# Autodesk Inventor assembly: CycloidalGearBoxAssemblyV1
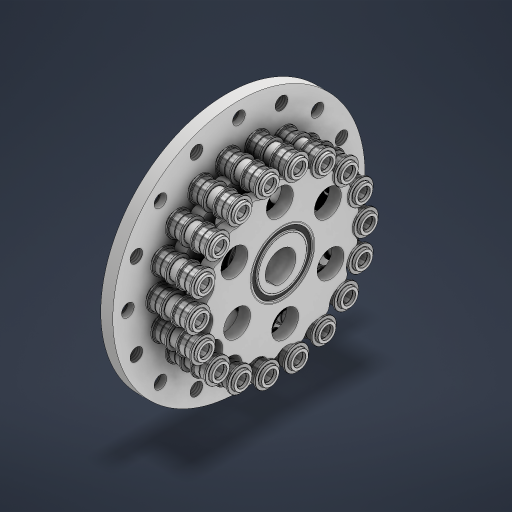
[picture p0: Inventor's stored thumbnail of the model, 512x512]
Saved by Autodesk Inventor 2024 (Build 280153000, 153)
## iProperties
Created: 2024-01-31
Part Number: CycloidalGearBoxAssemblyV1
Document SubType Name: Assembly
Designer: avsar
Author: avsar
## Documents named in this file (10)
- C:\Users\avsar\Documents\Inventor\RCR_Arm\Arm_V4\CycloidalGearBoxes\StageOneGearBox\CycloidalGearBoxAssemblyV1.iam
- C:\Users\avsar\Documents\Inventor\RCR_Arm\Arm_V4\CycloidalGearBoxes\StageOneGearBox\HousingFaceInput.ipt
- C:\Users\avsar\Documents\Inventor\RCR_Arm\Arm_V4\CycloidalGearBoxes\StageOneGearBox\Gearbox_MainBody.ipt
- C:\Users\avsar\Documents\Inventor\RCR_Arm\COTS\Motion\Bearings\Flanged Bearings\4x7x2.5mm Flanged Ball Bearing.ipt
- C:\Users\avsar\Documents\Inventor\RCR_Arm\COTS\ISO Standard Hardware\Spacers and Shims\4mm ID x 6mm OD Spacers\(1mm legnth) 4mm ID x 6mm OD Spacer.ipt
- C:\Users\avsar\Documents\Inventor\RCR_Arm\COTS\ISO Standard Hardware\Spacers and Shims\4mm ID x 6mm OD Spacers\(3mm legnth) 4mm ID x 6mm OD Spacer.ipt
- C:\Users\avsar\Documents\Inventor\RCR_Arm\Arm_V4\CycloidalGearBoxes\StageOneGearBox\RollerBearingShaft.ipt
- C:\Users\avsar\Documents\Inventor\RCR_Arm\Arm_V4\CycloidalGearBoxes\StageOneGearBox\CycloidalDisk.ipt
- C:\Users\avsar\Documents\Inventor\RCR_Arm\Arm_V4\CycloidalGearBoxes\StageOneGearBox\EccentricBearingShaft.ipt
- C:\Users\avsar\Documents\Inventor\RCR_Arm\COTS\Motion\Bearings\Standard Bearings\16mm ID x 22mm OD x 4mm Thickness Ball Bearing.ipt
## Components (169 placed, 9 different names)
1. HousingFaceInput:1 — Mate:1, Mate:2, Mate:3, Mate:4, Mate:5, Mate:7, Mate:75, Mate:76, Mate:93, Mate:94, Mate:111, Mate:112, Mate:129, Mate:130, Mate:147, Mate:148, Mate:165, Mate:166, Mate:183, Mate:184, Mate:201, Mate:202, Mate:219, Mate:220, Mate:237, Mate:238, Mate:255, Mate:256, Mate:273, Mate:274, Mate:291, Mate:292, Mate:309, Mate:310, Mate:327, Mate:328, Mate:345, Mate:346, Mate:363, Mate:364
2. Gearbox_MainBody:1 — Mate:1, Mate:2, Mate:3
3. (1mm legnth) 4mm ID x 6mm OD Spacer:1 — Mate:4, Mate:5, Mate:6, Mate:58
4. 4x7x2.5mm Flanged Ball Bearing:5 — Mate:10, Mate:11, Mate:12, Mate:13
5. RollerBearingShaft:2 — Mate:8, Mate:9, Mate:10, Mate:11
6. 4x7x2.5mm Flanged Ball Bearing:4 — Mate:6, Mate:7, Mate:8, Mate:9, Mate:58
7. (1mm legnth) 4mm ID x 6mm OD Spacer:2 — Mate:20, Mate:21
8. RollerBearingShaft:1 — Mate:16, Mate:17, Mate:18, Mate:19
9. 4x7x2.5mm Flanged Ball Bearing:2 — Mate:14, Mate:15, Mate:16, Mate:17
10. (3mm legnth) 4mm ID x 6mm OD Spacer:1 — Mate:12, Mate:13, Mate:14, Mate:15
11. 4x7x2.5mm Flanged Ball Bearing:1 — Mate:18, Mate:19, Mate:20, Mate:21
12. (1mm legnth) 4mm ID x 6mm OD Spacer:3 — Mate:76
13. (1mm legnth) 4mm ID x 6mm OD Spacer:4 — Mate:75
14. 4x7x2.5mm Flanged Ball Bearing:6
15. RollerBearingShaft:3
16. 4x7x2.5mm Flanged Ball Bearing:7 — Tangent:2
17. 4x7x2.5mm Flanged Ball Bearing:8
18. RollerBearingShaft:4
19. 4x7x2.5mm Flanged Ball Bearing:9
20. (3mm legnth) 4mm ID x 6mm OD Spacer:2
21. (1mm legnth) 4mm ID x 6mm OD Spacer:5 — Mate:94
22. (1mm legnth) 4mm ID x 6mm OD Spacer:6 — Mate:93
23. 4x7x2.5mm Flanged Ball Bearing:10
24. RollerBearingShaft:5
25. 4x7x2.5mm Flanged Ball Bearing:11
26. 4x7x2.5mm Flanged Ball Bearing:12
27. RollerBearingShaft:6
28. 4x7x2.5mm Flanged Ball Bearing:13
29. (3mm legnth) 4mm ID x 6mm OD Spacer:3
30. (1mm legnth) 4mm ID x 6mm OD Spacer:7 — Mate:112
31. (1mm legnth) 4mm ID x 6mm OD Spacer:8 — Mate:111
32. 4x7x2.5mm Flanged Ball Bearing:14
33. RollerBearingShaft:7
34. 4x7x2.5mm Flanged Ball Bearing:15
35. 4x7x2.5mm Flanged Ball Bearing:16 — Tangent:3
36. RollerBearingShaft:8
37. 4x7x2.5mm Flanged Ball Bearing:17
38. (3mm legnth) 4mm ID x 6mm OD Spacer:4
39. (1mm legnth) 4mm ID x 6mm OD Spacer:9
40. (1mm legnth) 4mm ID x 6mm OD Spacer:10 — Mate:129
41. 4x7x2.5mm Flanged Ball Bearing:18
42. RollerBearingShaft:9
43. 4x7x2.5mm Flanged Ball Bearing:19
44. 4x7x2.5mm Flanged Ball Bearing:20 — Mate:130
45. RollerBearingShaft:10
46. 4x7x2.5mm Flanged Ball Bearing:21
47. (3mm legnth) 4mm ID x 6mm OD Spacer:5
48. (1mm legnth) 4mm ID x 6mm OD Spacer:11
49. (1mm legnth) 4mm ID x 6mm OD Spacer:12 — Mate:147
50. 4x7x2.5mm Flanged Ball Bearing:22 — Mate:365, Tangent:1
51. RollerBearingShaft:11
52. 4x7x2.5mm Flanged Ball Bearing:23
53. 4x7x2.5mm Flanged Ball Bearing:24 — Mate:148
54. RollerBearingShaft:12
55. 4x7x2.5mm Flanged Ball Bearing:25 — Mate:366
56. (3mm legnth) 4mm ID x 6mm OD Spacer:6
57. (1mm legnth) 4mm ID x 6mm OD Spacer:13
58. (1mm legnth) 4mm ID x 6mm OD Spacer:14 — Mate:165
59. 4x7x2.5mm Flanged Ball Bearing:26
60. RollerBearingShaft:13
61. 4x7x2.5mm Flanged Ball Bearing:27
62. 4x7x2.5mm Flanged Ball Bearing:28 — Mate:166
63. RollerBearingShaft:14
64. 4x7x2.5mm Flanged Ball Bearing:29
65. (3mm legnth) 4mm ID x 6mm OD Spacer:7
66. (1mm legnth) 4mm ID x 6mm OD Spacer:15
67. (1mm legnth) 4mm ID x 6mm OD Spacer:16 — Mate:183
68. 4x7x2.5mm Flanged Ball Bearing:30
69. RollerBearingShaft:15
70. 4x7x2.5mm Flanged Ball Bearing:31
71. 4x7x2.5mm Flanged Ball Bearing:32 — Mate:184
72. RollerBearingShaft:16
73. 4x7x2.5mm Flanged Ball Bearing:33
74. (3mm legnth) 4mm ID x 6mm OD Spacer:8
75. (1mm legnth) 4mm ID x 6mm OD Spacer:17
76. (1mm legnth) 4mm ID x 6mm OD Spacer:18 — Mate:201
77. 4x7x2.5mm Flanged Ball Bearing:34
78. RollerBearingShaft:17
79. 4x7x2.5mm Flanged Ball Bearing:35
80. 4x7x2.5mm Flanged Ball Bearing:36 — Mate:202
81. RollerBearingShaft:18
82. 4x7x2.5mm Flanged Ball Bearing:37
83. (3mm legnth) 4mm ID x 6mm OD Spacer:9
84. (1mm legnth) 4mm ID x 6mm OD Spacer:19
85. (1mm legnth) 4mm ID x 6mm OD Spacer:20 — Mate:219
86. 4x7x2.5mm Flanged Ball Bearing:38
87. RollerBearingShaft:19
88. 4x7x2.5mm Flanged Ball Bearing:39
89. 4x7x2.5mm Flanged Ball Bearing:40 — Mate:220
90. RollerBearingShaft:20
91. 4x7x2.5mm Flanged Ball Bearing:41
92. (3mm legnth) 4mm ID x 6mm OD Spacer:10
93. (1mm legnth) 4mm ID x 6mm OD Spacer:21
94. (1mm legnth) 4mm ID x 6mm OD Spacer:22 — Mate:237
95. 4x7x2.5mm Flanged Ball Bearing:42
96. RollerBearingShaft:21
97. 4x7x2.5mm Flanged Ball Bearing:43
98. 4x7x2.5mm Flanged Ball Bearing:44 — Mate:238
99. RollerBearingShaft:22
100. 4x7x2.5mm Flanged Ball Bearing:45
101. (3mm legnth) 4mm ID x 6mm OD Spacer:11
102. (1mm legnth) 4mm ID x 6mm OD Spacer:23
103. (1mm legnth) 4mm ID x 6mm OD Spacer:24 — Mate:255
104. 4x7x2.5mm Flanged Ball Bearing:46 — Mate:256
105. RollerBearingShaft:23
106. 4x7x2.5mm Flanged Ball Bearing:47
107. 4x7x2.5mm Flanged Ball Bearing:48
108. RollerBearingShaft:24
109. 4x7x2.5mm Flanged Ball Bearing:49
110. (3mm legnth) 4mm ID x 6mm OD Spacer:12
111. (1mm legnth) 4mm ID x 6mm OD Spacer:25
112. (1mm legnth) 4mm ID x 6mm OD Spacer:26 — Mate:273
113. 4x7x2.5mm Flanged Ball Bearing:50
114. RollerBearingShaft:25
115. 4x7x2.5mm Flanged Ball Bearing:51
116. 4x7x2.5mm Flanged Ball Bearing:52 — Mate:274
117. RollerBearingShaft:26
118. 4x7x2.5mm Flanged Ball Bearing:53
119. (3mm legnth) 4mm ID x 6mm OD Spacer:13
120. (1mm legnth) 4mm ID x 6mm OD Spacer:27
121. (1mm legnth) 4mm ID x 6mm OD Spacer:28 — Mate:291
122. 4x7x2.5mm Flanged Ball Bearing:54
123. RollerBearingShaft:27
124. 4x7x2.5mm Flanged Ball Bearing:55
125. 4x7x2.5mm Flanged Ball Bearing:56 — Mate:292
126. RollerBearingShaft:28
127. 4x7x2.5mm Flanged Ball Bearing:57
128. (3mm legnth) 4mm ID x 6mm OD Spacer:14
129. (1mm legnth) 4mm ID x 6mm OD Spacer:29
130. (1mm legnth) 4mm ID x 6mm OD Spacer:30 — Mate:309
131. 4x7x2.5mm Flanged Ball Bearing:58
132. RollerBearingShaft:29
133. 4x7x2.5mm Flanged Ball Bearing:59
134. 4x7x2.5mm Flanged Ball Bearing:60 — Mate:310
135. RollerBearingShaft:30
136. 4x7x2.5mm Flanged Ball Bearing:61
137. (3mm legnth) 4mm ID x 6mm OD Spacer:15
138. (1mm legnth) 4mm ID x 6mm OD Spacer:31
139. (1mm legnth) 4mm ID x 6mm OD Spacer:32 — Mate:327
140. 4x7x2.5mm Flanged Ball Bearing:62
141. RollerBearingShaft:31
142. 4x7x2.5mm Flanged Ball Bearing:63
143. 4x7x2.5mm Flanged Ball Bearing:64 — Mate:328
144. RollerBearingShaft:32
145. 4x7x2.5mm Flanged Ball Bearing:65
146. (3mm legnth) 4mm ID x 6mm OD Spacer:16
147. (1mm legnth) 4mm ID x 6mm OD Spacer:33
148. (1mm legnth) 4mm ID x 6mm OD Spacer:34 — Mate:345
149. 4x7x2.5mm Flanged Ball Bearing:66
150. RollerBearingShaft:33
151. 4x7x2.5mm Flanged Ball Bearing:67
152. 4x7x2.5mm Flanged Ball Bearing:68 — Mate:346, Tangent:4
153. RollerBearingShaft:34
154. 4x7x2.5mm Flanged Ball Bearing:69
155. (3mm legnth) 4mm ID x 6mm OD Spacer:17
156. (1mm legnth) 4mm ID x 6mm OD Spacer:35
157. (1mm legnth) 4mm ID x 6mm OD Spacer:36 — Mate:363
158. 4x7x2.5mm Flanged Ball Bearing:70
159. RollerBearingShaft:35
160. 4x7x2.5mm Flanged Ball Bearing:71
161. 4x7x2.5mm Flanged Ball Bearing:72 — Mate:364
162. RollerBearingShaft:36
163. 4x7x2.5mm Flanged Ball Bearing:73
164. (3mm legnth) 4mm ID x 6mm OD Spacer:18
165. CycloidalDisk:1 — Mate:365, Tangent:1, Flush:2, Mate:368, Tangent:2
166. CycloidalDisk:2 — Mate:366, Flush:1, Mate:367, Tangent:3, Tangent:4
167. 16mm ID x 22mm OD x 4mm Thickness Ball Bearing:1 — Flush:1, Mate:367, Mate:370
168. 16mm ID x 22mm OD x 4mm Thickness Ball Bearing:2 — Flush:2, Mate:368, Flush:3, Mate:369
169. EccentricBearingShaft:1 — Flush:3, Mate:369, Mate:370
## Relationships (341: Mate 334, Tangent 4, Flush 3)
- Mate:1: HousingFaceInput:1 ↔ Gearbox_MainBody:1
- Mate:2: HousingFaceInput:1 ↔ Gearbox_MainBody:1
- Mate:3: HousingFaceInput:1 ↔ Gearbox_MainBody:1
- Mate:4: HousingFaceInput:1 ↔ (1mm legnth) 4mm ID x 6mm OD Spacer:1
- Mate:5: HousingFaceInput:1 ↔ (1mm legnth) 4mm ID x 6mm OD Spacer:1
- Mate:6: (1mm legnth) 4mm ID x 6mm OD Spacer:1 ↔ 4x7x2.5mm Flanged Ball Bearing:4
- Mate:7: HousingFaceInput:1 ↔ 4x7x2.5mm Flanged Ball Bearing:4
- Mate:8: RollerBearingShaft:2 ↔ 4x7x2.5mm Flanged Ball Bearing:4
- Mate:9: RollerBearingShaft:2 ↔ 4x7x2.5mm Flanged Ball Bearing:4
- Mate:10: 4x7x2.5mm Flanged Ball Bearing:5 ↔ RollerBearingShaft:2
- Mate:11: 4x7x2.5mm Flanged Ball Bearing:5 ↔ RollerBearingShaft:2
- Mate:12: 4x7x2.5mm Flanged Ball Bearing:5 ↔ (3mm legnth) 4mm ID x 6mm OD Spacer:1
- Mate:13: 4x7x2.5mm Flanged Ball Bearing:5 ↔ (3mm legnth) 4mm ID x 6mm OD Spacer:1
- Mate:14: 4x7x2.5mm Flanged Ball Bearing:2 ↔ (3mm legnth) 4mm ID x 6mm OD Spacer:1
- Mate:15: 4x7x2.5mm Flanged Ball Bearing:2 ↔ (3mm legnth) 4mm ID x 6mm OD Spacer:1
- Mate:16: RollerBearingShaft:1 ↔ 4x7x2.5mm Flanged Ball Bearing:2
- Mate:17: RollerBearingShaft:1 ↔ 4x7x2.5mm Flanged Ball Bearing:2
- Mate:18: RollerBearingShaft:1 ↔ 4x7x2.5mm Flanged Ball Bearing:1
- Mate:19: RollerBearingShaft:1 ↔ 4x7x2.5mm Flanged Ball Bearing:1
- Mate:20: (1mm legnth) 4mm ID x 6mm OD Spacer:2 ↔ 4x7x2.5mm Flanged Ball Bearing:1
- Mate:21: (1mm legnth) 4mm ID x 6mm OD Spacer:2 ↔ 4x7x2.5mm Flanged Ball Bearing:1
- Mate:58: (1mm legnth) 4mm ID x 6mm OD Spacer:1 ↔ 4x7x2.5mm Flanged Ball Bearing:4
- [Mate]: (1mm legnth) 4mm ID x 6mm OD Spacer:3 ↔ 4x7x2.5mm Flanged Ball Bearing:8
- [Mate]: 4x7x2.5mm Flanged Ball Bearing:8 ↔ RollerBearingShaft:4
- [Mate]: 4x7x2.5mm Flanged Ball Bearing:8 ↔ RollerBearingShaft:4
- [Mate]: RollerBearingShaft:4 ↔ 4x7x2.5mm Flanged Ball Bearing:9
- [Mate]: RollerBearingShaft:4 ↔ 4x7x2.5mm Flanged Ball Bearing:9
- [Mate]: 4x7x2.5mm Flanged Ball Bearing:9 ↔ (3mm legnth) 4mm ID x 6mm OD Spacer:2
- [Mate]: 4x7x2.5mm Flanged Ball Bearing:9 ↔ (3mm legnth) 4mm ID x 6mm OD Spacer:2
- [Mate]: 4x7x2.5mm Flanged Ball Bearing:7 ↔ (3mm legnth) 4mm ID x 6mm OD Spacer:2
- [Mate]: 4x7x2.5mm Flanged Ball Bearing:7 ↔ (3mm legnth) 4mm ID x 6mm OD Spacer:2
- [Mate]: RollerBearingShaft:3 ↔ 4x7x2.5mm Flanged Ball Bearing:7
- [Mate]: RollerBearingShaft:3 ↔ 4x7x2.5mm Flanged Ball Bearing:7
- [Mate]: 4x7x2.5mm Flanged Ball Bearing:6 ↔ RollerBearingShaft:3
- [Mate]: 4x7x2.5mm Flanged Ball Bearing:6 ↔ RollerBearingShaft:3
- [Mate]: (1mm legnth) 4mm ID x 6mm OD Spacer:4 ↔ 4x7x2.5mm Flanged Ball Bearing:6
- [Mate]: (1mm legnth) 4mm ID x 6mm OD Spacer:4 ↔ 4x7x2.5mm Flanged Ball Bearing:6
- [Mate]: (1mm legnth) 4mm ID x 6mm OD Spacer:3 ↔ 4x7x2.5mm Flanged Ball Bearing:8
- Mate:75: HousingFaceInput:1 ↔ (1mm legnth) 4mm ID x 6mm OD Spacer:4
- Mate:76: HousingFaceInput:1 ↔ (1mm legnth) 4mm ID x 6mm OD Spacer:3
- [Mate]: (1mm legnth) 4mm ID x 6mm OD Spacer:5 ↔ 4x7x2.5mm Flanged Ball Bearing:12
- [Mate]: 4x7x2.5mm Flanged Ball Bearing:12 ↔ RollerBearingShaft:6
- [Mate]: 4x7x2.5mm Flanged Ball Bearing:12 ↔ RollerBearingShaft:6
- [Mate]: RollerBearingShaft:6 ↔ 4x7x2.5mm Flanged Ball Bearing:13
- [Mate]: RollerBearingShaft:6 ↔ 4x7x2.5mm Flanged Ball Bearing:13
- [Mate]: 4x7x2.5mm Flanged Ball Bearing:13 ↔ (3mm legnth) 4mm ID x 6mm OD Spacer:3
- [Mate]: 4x7x2.5mm Flanged Ball Bearing:13 ↔ (3mm legnth) 4mm ID x 6mm OD Spacer:3
- [Mate]: 4x7x2.5mm Flanged Ball Bearing:11 ↔ (3mm legnth) 4mm ID x 6mm OD Spacer:3
- [Mate]: 4x7x2.5mm Flanged Ball Bearing:11 ↔ (3mm legnth) 4mm ID x 6mm OD Spacer:3
- [Mate]: RollerBearingShaft:5 ↔ 4x7x2.5mm Flanged Ball Bearing:11
- [Mate]: RollerBearingShaft:5 ↔ 4x7x2.5mm Flanged Ball Bearing:11
- [Mate]: 4x7x2.5mm Flanged Ball Bearing:10 ↔ RollerBearingShaft:5
- [Mate]: 4x7x2.5mm Flanged Ball Bearing:10 ↔ RollerBearingShaft:5
- [Mate]: (1mm legnth) 4mm ID x 6mm OD Spacer:6 ↔ 4x7x2.5mm Flanged Ball Bearing:10
- [Mate]: (1mm legnth) 4mm ID x 6mm OD Spacer:6 ↔ 4x7x2.5mm Flanged Ball Bearing:10
- [Mate]: (1mm legnth) 4mm ID x 6mm OD Spacer:5 ↔ 4x7x2.5mm Flanged Ball Bearing:12
- Mate:93: HousingFaceInput:1 ↔ (1mm legnth) 4mm ID x 6mm OD Spacer:6
- Mate:94: HousingFaceInput:1 ↔ (1mm legnth) 4mm ID x 6mm OD Spacer:5
- [Mate]: (1mm legnth) 4mm ID x 6mm OD Spacer:7 ↔ 4x7x2.5mm Flanged Ball Bearing:16
- [Mate]: 4x7x2.5mm Flanged Ball Bearing:16 ↔ RollerBearingShaft:8
- [Mate]: 4x7x2.5mm Flanged Ball Bearing:16 ↔ RollerBearingShaft:8
- [Mate]: RollerBearingShaft:8 ↔ 4x7x2.5mm Flanged Ball Bearing:17
- [Mate]: RollerBearingShaft:8 ↔ 4x7x2.5mm Flanged Ball Bearing:17
- [Mate]: 4x7x2.5mm Flanged Ball Bearing:17 ↔ (3mm legnth) 4mm ID x 6mm OD Spacer:4
- [Mate]: 4x7x2.5mm Flanged Ball Bearing:17 ↔ (3mm legnth) 4mm ID x 6mm OD Spacer:4
- [Mate]: 4x7x2.5mm Flanged Ball Bearing:15 ↔ (3mm legnth) 4mm ID x 6mm OD Spacer:4
- [Mate]: 4x7x2.5mm Flanged Ball Bearing:15 ↔ (3mm legnth) 4mm ID x 6mm OD Spacer:4
- [Mate]: RollerBearingShaft:7 ↔ 4x7x2.5mm Flanged Ball Bearing:15
- [Mate]: RollerBearingShaft:7 ↔ 4x7x2.5mm Flanged Ball Bearing:15
- [Mate]: 4x7x2.5mm Flanged Ball Bearing:14 ↔ RollerBearingShaft:7
- [Mate]: 4x7x2.5mm Flanged Ball Bearing:14 ↔ RollerBearingShaft:7
- [Mate]: (1mm legnth) 4mm ID x 6mm OD Spacer:8 ↔ 4x7x2.5mm Flanged Ball Bearing:14
- [Mate]: (1mm legnth) 4mm ID x 6mm OD Spacer:8 ↔ 4x7x2.5mm Flanged Ball Bearing:14
- [Mate]: (1mm legnth) 4mm ID x 6mm OD Spacer:7 ↔ 4x7x2.5mm Flanged Ball Bearing:16
- Mate:111: HousingFaceInput:1 ↔ (1mm legnth) 4mm ID x 6mm OD Spacer:8
- Mate:112: HousingFaceInput:1 ↔ (1mm legnth) 4mm ID x 6mm OD Spacer:7
- [Mate]: (1mm legnth) 4mm ID x 6mm OD Spacer:9 ↔ 4x7x2.5mm Flanged Ball Bearing:20
- [Mate]: 4x7x2.5mm Flanged Ball Bearing:20 ↔ RollerBearingShaft:10
- [Mate]: 4x7x2.5mm Flanged Ball Bearing:20 ↔ RollerBearingShaft:10
- [Mate]: RollerBearingShaft:10 ↔ 4x7x2.5mm Flanged Ball Bearing:21
- [Mate]: RollerBearingShaft:10 ↔ 4x7x2.5mm Flanged Ball Bearing:21
- [Mate]: 4x7x2.5mm Flanged Ball Bearing:21 ↔ (3mm legnth) 4mm ID x 6mm OD Spacer:5
- [Mate]: 4x7x2.5mm Flanged Ball Bearing:21 ↔ (3mm legnth) 4mm ID x 6mm OD Spacer:5
- [Mate]: 4x7x2.5mm Flanged Ball Bearing:19 ↔ (3mm legnth) 4mm ID x 6mm OD Spacer:5
- [Mate]: 4x7x2.5mm Flanged Ball Bearing:19 ↔ (3mm legnth) 4mm ID x 6mm OD Spacer:5
- [Mate]: RollerBearingShaft:9 ↔ 4x7x2.5mm Flanged Ball Bearing:19
- [Mate]: RollerBearingShaft:9 ↔ 4x7x2.5mm Flanged Ball Bearing:19
- [Mate]: 4x7x2.5mm Flanged Ball Bearing:18 ↔ RollerBearingShaft:9
- [Mate]: 4x7x2.5mm Flanged Ball Bearing:18 ↔ RollerBearingShaft:9
- [Mate]: (1mm legnth) 4mm ID x 6mm OD Spacer:10 ↔ 4x7x2.5mm Flanged Ball Bearing:18
- [Mate]: (1mm legnth) 4mm ID x 6mm OD Spacer:10 ↔ 4x7x2.5mm Flanged Ball Bearing:18
- [Mate]: (1mm legnth) 4mm ID x 6mm OD Spacer:9 ↔ 4x7x2.5mm Flanged Ball Bearing:20
- Mate:129: HousingFaceInput:1 ↔ (1mm legnth) 4mm ID x 6mm OD Spacer:10
- Mate:130: HousingFaceInput:1 ↔ 4x7x2.5mm Flanged Ball Bearing:20
- [Mate]: (1mm legnth) 4mm ID x 6mm OD Spacer:11 ↔ 4x7x2.5mm Flanged Ball Bearing:24
- [Mate]: 4x7x2.5mm Flanged Ball Bearing:24 ↔ RollerBearingShaft:12
- [Mate]: 4x7x2.5mm Flanged Ball Bearing:24 ↔ RollerBearingShaft:12
- [Mate]: RollerBearingShaft:12 ↔ 4x7x2.5mm Flanged Ball Bearing:25
- [Mate]: RollerBearingShaft:12 ↔ 4x7x2.5mm Flanged Ball Bearing:25
- [Mate]: 4x7x2.5mm Flanged Ball Bearing:25 ↔ (3mm legnth) 4mm ID x 6mm OD Spacer:6
- [Mate]: 4x7x2.5mm Flanged Ball Bearing:25 ↔ (3mm legnth) 4mm ID x 6mm OD Spacer:6
- [Mate]: 4x7x2.5mm Flanged Ball Bearing:23 ↔ (3mm legnth) 4mm ID x 6mm OD Spacer:6
- [Mate]: 4x7x2.5mm Flanged Ball Bearing:23 ↔ (3mm legnth) 4mm ID x 6mm OD Spacer:6
- [Mate]: RollerBearingShaft:11 ↔ 4x7x2.5mm Flanged Ball Bearing:23
- [Mate]: RollerBearingShaft:11 ↔ 4x7x2.5mm Flanged Ball Bearing:23
- [Mate]: 4x7x2.5mm Flanged Ball Bearing:22 ↔ RollerBearingShaft:11
- [Mate]: 4x7x2.5mm Flanged Ball Bearing:22 ↔ RollerBearingShaft:11
- [Mate]: (1mm legnth) 4mm ID x 6mm OD Spacer:12 ↔ 4x7x2.5mm Flanged Ball Bearing:22
- [Mate]: (1mm legnth) 4mm ID x 6mm OD Spacer:12 ↔ 4x7x2.5mm Flanged Ball Bearing:22
- [Mate]: (1mm legnth) 4mm ID x 6mm OD Spacer:11 ↔ 4x7x2.5mm Flanged Ball Bearing:24
- Mate:147: HousingFaceInput:1 ↔ (1mm legnth) 4mm ID x 6mm OD Spacer:12
- Mate:148: HousingFaceInput:1 ↔ 4x7x2.5mm Flanged Ball Bearing:24
- [Mate]: (1mm legnth) 4mm ID x 6mm OD Spacer:13 ↔ 4x7x2.5mm Flanged Ball Bearing:28
- [Mate]: 4x7x2.5mm Flanged Ball Bearing:28 ↔ RollerBearingShaft:14
- [Mate]: 4x7x2.5mm Flanged Ball Bearing:28 ↔ RollerBearingShaft:14
- [Mate]: RollerBearingShaft:14 ↔ 4x7x2.5mm Flanged Ball Bearing:29
- [Mate]: RollerBearingShaft:14 ↔ 4x7x2.5mm Flanged Ball Bearing:29
- [Mate]: 4x7x2.5mm Flanged Ball Bearing:29 ↔ (3mm legnth) 4mm ID x 6mm OD Spacer:7
- [Mate]: 4x7x2.5mm Flanged Ball Bearing:29 ↔ (3mm legnth) 4mm ID x 6mm OD Spacer:7
- [Mate]: 4x7x2.5mm Flanged Ball Bearing:27 ↔ (3mm legnth) 4mm ID x 6mm OD Spacer:7
- [Mate]: 4x7x2.5mm Flanged Ball Bearing:27 ↔ (3mm legnth) 4mm ID x 6mm OD Spacer:7
- [Mate]: RollerBearingShaft:13 ↔ 4x7x2.5mm Flanged Ball Bearing:27
- [Mate]: RollerBearingShaft:13 ↔ 4x7x2.5mm Flanged Ball Bearing:27
- [Mate]: 4x7x2.5mm Flanged Ball Bearing:26 ↔ RollerBearingShaft:13
- [Mate]: 4x7x2.5mm Flanged Ball Bearing:26 ↔ RollerBearingShaft:13
- [Mate]: (1mm legnth) 4mm ID x 6mm OD Spacer:14 ↔ 4x7x2.5mm Flanged Ball Bearing:26
- [Mate]: (1mm legnth) 4mm ID x 6mm OD Spacer:14 ↔ 4x7x2.5mm Flanged Ball Bearing:26
- [Mate]: (1mm legnth) 4mm ID x 6mm OD Spacer:13 ↔ 4x7x2.5mm Flanged Ball Bearing:28
- Mate:165: HousingFaceInput:1 ↔ (1mm legnth) 4mm ID x 6mm OD Spacer:14
- Mate:166: HousingFaceInput:1 ↔ 4x7x2.5mm Flanged Ball Bearing:28
- [Mate]: (1mm legnth) 4mm ID x 6mm OD Spacer:15 ↔ 4x7x2.5mm Flanged Ball Bearing:32
- [Mate]: 4x7x2.5mm Flanged Ball Bearing:32 ↔ RollerBearingShaft:16
- [Mate]: 4x7x2.5mm Flanged Ball Bearing:32 ↔ RollerBearingShaft:16
- [Mate]: RollerBearingShaft:16 ↔ 4x7x2.5mm Flanged Ball Bearing:33
- [Mate]: RollerBearingShaft:16 ↔ 4x7x2.5mm Flanged Ball Bearing:33
- [Mate]: 4x7x2.5mm Flanged Ball Bearing:33 ↔ (3mm legnth) 4mm ID x 6mm OD Spacer:8
- [Mate]: 4x7x2.5mm Flanged Ball Bearing:33 ↔ (3mm legnth) 4mm ID x 6mm OD Spacer:8
- [Mate]: 4x7x2.5mm Flanged Ball Bearing:31 ↔ (3mm legnth) 4mm ID x 6mm OD Spacer:8
- [Mate]: 4x7x2.5mm Flanged Ball Bearing:31 ↔ (3mm legnth) 4mm ID x 6mm OD Spacer:8
- [Mate]: RollerBearingShaft:15 ↔ 4x7x2.5mm Flanged Ball Bearing:31
- [Mate]: RollerBearingShaft:15 ↔ 4x7x2.5mm Flanged Ball Bearing:31
- [Mate]: 4x7x2.5mm Flanged Ball Bearing:30 ↔ RollerBearingShaft:15
- [Mate]: 4x7x2.5mm Flanged Ball Bearing:30 ↔ RollerBearingShaft:15
- [Mate]: (1mm legnth) 4mm ID x 6mm OD Spacer:16 ↔ 4x7x2.5mm Flanged Ball Bearing:30
- [Mate]: (1mm legnth) 4mm ID x 6mm OD Spacer:16 ↔ 4x7x2.5mm Flanged Ball Bearing:30
- [Mate]: (1mm legnth) 4mm ID x 6mm OD Spacer:15 ↔ 4x7x2.5mm Flanged Ball Bearing:32
- Mate:183: HousingFaceInput:1 ↔ (1mm legnth) 4mm ID x 6mm OD Spacer:16
- Mate:184: HousingFaceInput:1 ↔ 4x7x2.5mm Flanged Ball Bearing:32
- [Mate]: (1mm legnth) 4mm ID x 6mm OD Spacer:17 ↔ 4x7x2.5mm Flanged Ball Bearing:36
- [Mate]: 4x7x2.5mm Flanged Ball Bearing:36 ↔ RollerBearingShaft:18
- [Mate]: 4x7x2.5mm Flanged Ball Bearing:36 ↔ RollerBearingShaft:18
- [Mate]: RollerBearingShaft:18 ↔ 4x7x2.5mm Flanged Ball Bearing:37
- [Mate]: RollerBearingShaft:18 ↔ 4x7x2.5mm Flanged Ball Bearing:37
- [Mate]: 4x7x2.5mm Flanged Ball Bearing:37 ↔ (3mm legnth) 4mm ID x 6mm OD Spacer:9
- [Mate]: 4x7x2.5mm Flanged Ball Bearing:37 ↔ (3mm legnth) 4mm ID x 6mm OD Spacer:9
- [Mate]: 4x7x2.5mm Flanged Ball Bearing:35 ↔ (3mm legnth) 4mm ID x 6mm OD Spacer:9
- [Mate]: 4x7x2.5mm Flanged Ball Bearing:35 ↔ (3mm legnth) 4mm ID x 6mm OD Spacer:9
- [Mate]: RollerBearingShaft:17 ↔ 4x7x2.5mm Flanged Ball Bearing:35
- [Mate]: RollerBearingShaft:17 ↔ 4x7x2.5mm Flanged Ball Bearing:35
- [Mate]: 4x7x2.5mm Flanged Ball Bearing:34 ↔ RollerBearingShaft:17
- [Mate]: 4x7x2.5mm Flanged Ball Bearing:34 ↔ RollerBearingShaft:17
- [Mate]: (1mm legnth) 4mm ID x 6mm OD Spacer:18 ↔ 4x7x2.5mm Flanged Ball Bearing:34
- [Mate]: (1mm legnth) 4mm ID x 6mm OD Spacer:18 ↔ 4x7x2.5mm Flanged Ball Bearing:34
- [Mate]: (1mm legnth) 4mm ID x 6mm OD Spacer:17 ↔ 4x7x2.5mm Flanged Ball Bearing:36
- Mate:201: HousingFaceInput:1 ↔ (1mm legnth) 4mm ID x 6mm OD Spacer:18
- Mate:202: HousingFaceInput:1 ↔ 4x7x2.5mm Flanged Ball Bearing:36
- [Mate]: (1mm legnth) 4mm ID x 6mm OD Spacer:19 ↔ 4x7x2.5mm Flanged Ball Bearing:40
- [Mate]: 4x7x2.5mm Flanged Ball Bearing:40 ↔ RollerBearingShaft:20
- [Mate]: 4x7x2.5mm Flanged Ball Bearing:40 ↔ RollerBearingShaft:20
- [Mate]: RollerBearingShaft:20 ↔ 4x7x2.5mm Flanged Ball Bearing:41
- [Mate]: RollerBearingShaft:20 ↔ 4x7x2.5mm Flanged Ball Bearing:41
- [Mate]: 4x7x2.5mm Flanged Ball Bearing:41 ↔ (3mm legnth) 4mm ID x 6mm OD Spacer:10
- [Mate]: 4x7x2.5mm Flanged Ball Bearing:41 ↔ (3mm legnth) 4mm ID x 6mm OD Spacer:10
- [Mate]: 4x7x2.5mm Flanged Ball Bearing:39 ↔ (3mm legnth) 4mm ID x 6mm OD Spacer:10
- [Mate]: 4x7x2.5mm Flanged Ball Bearing:39 ↔ (3mm legnth) 4mm ID x 6mm OD Spacer:10
- [Mate]: RollerBearingShaft:19 ↔ 4x7x2.5mm Flanged Ball Bearing:39
- [Mate]: RollerBearingShaft:19 ↔ 4x7x2.5mm Flanged Ball Bearing:39
- [Mate]: 4x7x2.5mm Flanged Ball Bearing:38 ↔ RollerBearingShaft:19
- [Mate]: 4x7x2.5mm Flanged Ball Bearing:38 ↔ RollerBearingShaft:19
- [Mate]: (1mm legnth) 4mm ID x 6mm OD Spacer:20 ↔ 4x7x2.5mm Flanged Ball Bearing:38
- [Mate]: (1mm legnth) 4mm ID x 6mm OD Spacer:20 ↔ 4x7x2.5mm Flanged Ball Bearing:38
- [Mate]: (1mm legnth) 4mm ID x 6mm OD Spacer:19 ↔ 4x7x2.5mm Flanged Ball Bearing:40
- Mate:219: HousingFaceInput:1 ↔ (1mm legnth) 4mm ID x 6mm OD Spacer:20
- Mate:220: HousingFaceInput:1 ↔ 4x7x2.5mm Flanged Ball Bearing:40
- [Mate]: (1mm legnth) 4mm ID x 6mm OD Spacer:21 ↔ 4x7x2.5mm Flanged Ball Bearing:44
- [Mate]: 4x7x2.5mm Flanged Ball Bearing:44 ↔ RollerBearingShaft:22
- [Mate]: 4x7x2.5mm Flanged Ball Bearing:44 ↔ RollerBearingShaft:22
- [Mate]: RollerBearingShaft:22 ↔ 4x7x2.5mm Flanged Ball Bearing:45
- [Mate]: RollerBearingShaft:22 ↔ 4x7x2.5mm Flanged Ball Bearing:45
- [Mate]: 4x7x2.5mm Flanged Ball Bearing:45 ↔ (3mm legnth) 4mm ID x 6mm OD Spacer:11
- [Mate]: 4x7x2.5mm Flanged Ball Bearing:45 ↔ (3mm legnth) 4mm ID x 6mm OD Spacer:11
- [Mate]: 4x7x2.5mm Flanged Ball Bearing:43 ↔ (3mm legnth) 4mm ID x 6mm OD Spacer:11
- [Mate]: 4x7x2.5mm Flanged Ball Bearing:43 ↔ (3mm legnth) 4mm ID x 6mm OD Spacer:11
- [Mate]: RollerBearingShaft:21 ↔ 4x7x2.5mm Flanged Ball Bearing:43
- [Mate]: RollerBearingShaft:21 ↔ 4x7x2.5mm Flanged Ball Bearing:43
- [Mate]: 4x7x2.5mm Flanged Ball Bearing:42 ↔ RollerBearingShaft:21
- [Mate]: 4x7x2.5mm Flanged Ball Bearing:42 ↔ RollerBearingShaft:21
- [Mate]: (1mm legnth) 4mm ID x 6mm OD Spacer:22 ↔ 4x7x2.5mm Flanged Ball Bearing:42
- [Mate]: (1mm legnth) 4mm ID x 6mm OD Spacer:22 ↔ 4x7x2.5mm Flanged Ball Bearing:42
- [Mate]: (1mm legnth) 4mm ID x 6mm OD Spacer:21 ↔ 4x7x2.5mm Flanged Ball Bearing:44
- Mate:237: HousingFaceInput:1 ↔ (1mm legnth) 4mm ID x 6mm OD Spacer:22
- Mate:238: HousingFaceInput:1 ↔ 4x7x2.5mm Flanged Ball Bearing:44
- [Mate]: (1mm legnth) 4mm ID x 6mm OD Spacer:23 ↔ 4x7x2.5mm Flanged Ball Bearing:48
- [Mate]: 4x7x2.5mm Flanged Ball Bearing:48 ↔ RollerBearingShaft:24
- [Mate]: 4x7x2.5mm Flanged Ball Bearing:48 ↔ RollerBearingShaft:24
- [Mate]: RollerBearingShaft:24 ↔ 4x7x2.5mm Flanged Ball Bearing:49
- [Mate]: RollerBearingShaft:24 ↔ 4x7x2.5mm Flanged Ball Bearing:49
- [Mate]: 4x7x2.5mm Flanged Ball Bearing:49 ↔ (3mm legnth) 4mm ID x 6mm OD Spacer:12
- [Mate]: 4x7x2.5mm Flanged Ball Bearing:49 ↔ (3mm legnth) 4mm ID x 6mm OD Spacer:12
- [Mate]: 4x7x2.5mm Flanged Ball Bearing:47 ↔ (3mm legnth) 4mm ID x 6mm OD Spacer:12
- [Mate]: 4x7x2.5mm Flanged Ball Bearing:47 ↔ (3mm legnth) 4mm ID x 6mm OD Spacer:12
- [Mate]: RollerBearingShaft:23 ↔ 4x7x2.5mm Flanged Ball Bearing:47
- [Mate]: RollerBearingShaft:23 ↔ 4x7x2.5mm Flanged Ball Bearing:47
- [Mate]: 4x7x2.5mm Flanged Ball Bearing:46 ↔ RollerBearingShaft:23
- [Mate]: 4x7x2.5mm Flanged Ball Bearing:46 ↔ RollerBearingShaft:23
- [Mate]: (1mm legnth) 4mm ID x 6mm OD Spacer:24 ↔ 4x7x2.5mm Flanged Ball Bearing:46
- [Mate]: (1mm legnth) 4mm ID x 6mm OD Spacer:24 ↔ 4x7x2.5mm Flanged Ball Bearing:46
- [Mate]: (1mm legnth) 4mm ID x 6mm OD Spacer:23 ↔ 4x7x2.5mm Flanged Ball Bearing:48
- Mate:255: HousingFaceInput:1 ↔ (1mm legnth) 4mm ID x 6mm OD Spacer:24
- Mate:256: HousingFaceInput:1 ↔ 4x7x2.5mm Flanged Ball Bearing:46
- [Mate]: (1mm legnth) 4mm ID x 6mm OD Spacer:25 ↔ 4x7x2.5mm Flanged Ball Bearing:52
- [Mate]: 4x7x2.5mm Flanged Ball Bearing:52 ↔ RollerBearingShaft:26
- [Mate]: 4x7x2.5mm Flanged Ball Bearing:52 ↔ RollerBearingShaft:26
- [Mate]: RollerBearingShaft:26 ↔ 4x7x2.5mm Flanged Ball Bearing:53
- [Mate]: RollerBearingShaft:26 ↔ 4x7x2.5mm Flanged Ball Bearing:53
- [Mate]: 4x7x2.5mm Flanged Ball Bearing:53 ↔ (3mm legnth) 4mm ID x 6mm OD Spacer:13
- [Mate]: 4x7x2.5mm Flanged Ball Bearing:53 ↔ (3mm legnth) 4mm ID x 6mm OD Spacer:13
- [Mate]: 4x7x2.5mm Flanged Ball Bearing:51 ↔ (3mm legnth) 4mm ID x 6mm OD Spacer:13
- [Mate]: 4x7x2.5mm Flanged Ball Bearing:51 ↔ (3mm legnth) 4mm ID x 6mm OD Spacer:13
- [Mate]: RollerBearingShaft:25 ↔ 4x7x2.5mm Flanged Ball Bearing:51
- [Mate]: RollerBearingShaft:25 ↔ 4x7x2.5mm Flanged Ball Bearing:51
- [Mate]: 4x7x2.5mm Flanged Ball Bearing:50 ↔ RollerBearingShaft:25
- [Mate]: 4x7x2.5mm Flanged Ball Bearing:50 ↔ RollerBearingShaft:25
- [Mate]: (1mm legnth) 4mm ID x 6mm OD Spacer:26 ↔ 4x7x2.5mm Flanged Ball Bearing:50
- [Mate]: (1mm legnth) 4mm ID x 6mm OD Spacer:26 ↔ 4x7x2.5mm Flanged Ball Bearing:50
- [Mate]: (1mm legnth) 4mm ID x 6mm OD Spacer:25 ↔ 4x7x2.5mm Flanged Ball Bearing:52
- Mate:273: HousingFaceInput:1 ↔ (1mm legnth) 4mm ID x 6mm OD Spacer:26
- Mate:274: HousingFaceInput:1 ↔ 4x7x2.5mm Flanged Ball Bearing:52
- [Mate]: (1mm legnth) 4mm ID x 6mm OD Spacer:27 ↔ 4x7x2.5mm Flanged Ball Bearing:56
- [Mate]: 4x7x2.5mm Flanged Ball Bearing:56 ↔ RollerBearingShaft:28
- [Mate]: 4x7x2.5mm Flanged Ball Bearing:56 ↔ RollerBearingShaft:28
- [Mate]: RollerBearingShaft:28 ↔ 4x7x2.5mm Flanged Ball Bearing:57
- [Mate]: RollerBearingShaft:28 ↔ 4x7x2.5mm Flanged Ball Bearing:57
- [Mate]: 4x7x2.5mm Flanged Ball Bearing:57 ↔ (3mm legnth) 4mm ID x 6mm OD Spacer:14
- [Mate]: 4x7x2.5mm Flanged Ball Bearing:57 ↔ (3mm legnth) 4mm ID x 6mm OD Spacer:14
- [Mate]: 4x7x2.5mm Flanged Ball Bearing:55 ↔ (3mm legnth) 4mm ID x 6mm OD Spacer:14
- [Mate]: 4x7x2.5mm Flanged Ball Bearing:55 ↔ (3mm legnth) 4mm ID x 6mm OD Spacer:14
- [Mate]: RollerBearingShaft:27 ↔ 4x7x2.5mm Flanged Ball Bearing:55
- [Mate]: RollerBearingShaft:27 ↔ 4x7x2.5mm Flanged Ball Bearing:55
- [Mate]: 4x7x2.5mm Flanged Ball Bearing:54 ↔ RollerBearingShaft:27
- [Mate]: 4x7x2.5mm Flanged Ball Bearing:54 ↔ RollerBearingShaft:27
- [Mate]: (1mm legnth) 4mm ID x 6mm OD Spacer:28 ↔ 4x7x2.5mm Flanged Ball Bearing:54
- [Mate]: (1mm legnth) 4mm ID x 6mm OD Spacer:28 ↔ 4x7x2.5mm Flanged Ball Bearing:54
- [Mate]: (1mm legnth) 4mm ID x 6mm OD Spacer:27 ↔ 4x7x2.5mm Flanged Ball Bearing:56
- Mate:291: HousingFaceInput:1 ↔ (1mm legnth) 4mm ID x 6mm OD Spacer:28
- Mate:292: HousingFaceInput:1 ↔ 4x7x2.5mm Flanged Ball Bearing:56
- [Mate]: (1mm legnth) 4mm ID x 6mm OD Spacer:29 ↔ 4x7x2.5mm Flanged Ball Bearing:60
- [Mate]: 4x7x2.5mm Flanged Ball Bearing:60 ↔ RollerBearingShaft:30
- [Mate]: 4x7x2.5mm Flanged Ball Bearing:60 ↔ RollerBearingShaft:30
- [Mate]: RollerBearingShaft:30 ↔ 4x7x2.5mm Flanged Ball Bearing:61
- [Mate]: RollerBearingShaft:30 ↔ 4x7x2.5mm Flanged Ball Bearing:61
- [Mate]: 4x7x2.5mm Flanged Ball Bearing:61 ↔ (3mm legnth) 4mm ID x 6mm OD Spacer:15
- [Mate]: 4x7x2.5mm Flanged Ball Bearing:61 ↔ (3mm legnth) 4mm ID x 6mm OD Spacer:15
- [Mate]: 4x7x2.5mm Flanged Ball Bearing:59 ↔ (3mm legnth) 4mm ID x 6mm OD Spacer:15
- [Mate]: 4x7x2.5mm Flanged Ball Bearing:59 ↔ (3mm legnth) 4mm ID x 6mm OD Spacer:15
- [Mate]: RollerBearingShaft:29 ↔ 4x7x2.5mm Flanged Ball Bearing:59
- [Mate]: RollerBearingShaft:29 ↔ 4x7x2.5mm Flanged Ball Bearing:59
- [Mate]: 4x7x2.5mm Flanged Ball Bearing:58 ↔ RollerBearingShaft:29
- [Mate]: 4x7x2.5mm Flanged Ball Bearing:58 ↔ RollerBearingShaft:29
- [Mate]: (1mm legnth) 4mm ID x 6mm OD Spacer:30 ↔ 4x7x2.5mm Flanged Ball Bearing:58
- [Mate]: (1mm legnth) 4mm ID x 6mm OD Spacer:30 ↔ 4x7x2.5mm Flanged Ball Bearing:58
- [Mate]: (1mm legnth) 4mm ID x 6mm OD Spacer:29 ↔ 4x7x2.5mm Flanged Ball Bearing:60
- Mate:309: HousingFaceInput:1 ↔ (1mm legnth) 4mm ID x 6mm OD Spacer:30
- Mate:310: HousingFaceInput:1 ↔ 4x7x2.5mm Flanged Ball Bearing:60
- [Mate]: (1mm legnth) 4mm ID x 6mm OD Spacer:31 ↔ 4x7x2.5mm Flanged Ball Bearing:64
- [Mate]: 4x7x2.5mm Flanged Ball Bearing:64 ↔ RollerBearingShaft:32
- [Mate]: 4x7x2.5mm Flanged Ball Bearing:64 ↔ RollerBearingShaft:32
- [Mate]: RollerBearingShaft:32 ↔ 4x7x2.5mm Flanged Ball Bearing:65
- [Mate]: RollerBearingShaft:32 ↔ 4x7x2.5mm Flanged Ball Bearing:65
- [Mate]: 4x7x2.5mm Flanged Ball Bearing:65 ↔ (3mm legnth) 4mm ID x 6mm OD Spacer:16
- [Mate]: 4x7x2.5mm Flanged Ball Bearing:65 ↔ (3mm legnth) 4mm ID x 6mm OD Spacer:16
- [Mate]: 4x7x2.5mm Flanged Ball Bearing:63 ↔ (3mm legnth) 4mm ID x 6mm OD Spacer:16
- [Mate]: 4x7x2.5mm Flanged Ball Bearing:63 ↔ (3mm legnth) 4mm ID x 6mm OD Spacer:16
- [Mate]: RollerBearingShaft:31 ↔ 4x7x2.5mm Flanged Ball Bearing:63
- [Mate]: RollerBearingShaft:31 ↔ 4x7x2.5mm Flanged Ball Bearing:63
- [Mate]: 4x7x2.5mm Flanged Ball Bearing:62 ↔ RollerBearingShaft:31
- [Mate]: 4x7x2.5mm Flanged Ball Bearing:62 ↔ RollerBearingShaft:31
- [Mate]: (1mm legnth) 4mm ID x 6mm OD Spacer:32 ↔ 4x7x2.5mm Flanged Ball Bearing:62
- [Mate]: (1mm legnth) 4mm ID x 6mm OD Spacer:32 ↔ 4x7x2.5mm Flanged Ball Bearing:62
- [Mate]: (1mm legnth) 4mm ID x 6mm OD Spacer:31 ↔ 4x7x2.5mm Flanged Ball Bearing:64
- Mate:327: HousingFaceInput:1 ↔ (1mm legnth) 4mm ID x 6mm OD Spacer:32
- Mate:328: HousingFaceInput:1 ↔ 4x7x2.5mm Flanged Ball Bearing:64
- [Mate]: (1mm legnth) 4mm ID x 6mm OD Spacer:33 ↔ 4x7x2.5mm Flanged Ball Bearing:68
- [Mate]: 4x7x2.5mm Flanged Ball Bearing:68 ↔ RollerBearingShaft:34
- [Mate]: 4x7x2.5mm Flanged Ball Bearing:68 ↔ RollerBearingShaft:34
- [Mate]: RollerBearingShaft:34 ↔ 4x7x2.5mm Flanged Ball Bearing:69
- [Mate]: RollerBearingShaft:34 ↔ 4x7x2.5mm Flanged Ball Bearing:69
- [Mate]: 4x7x2.5mm Flanged Ball Bearing:69 ↔ (3mm legnth) 4mm ID x 6mm OD Spacer:17
- [Mate]: 4x7x2.5mm Flanged Ball Bearing:69 ↔ (3mm legnth) 4mm ID x 6mm OD Spacer:17
- [Mate]: 4x7x2.5mm Flanged Ball Bearing:67 ↔ (3mm legnth) 4mm ID x 6mm OD Spacer:17
- [Mate]: 4x7x2.5mm Flanged Ball Bearing:67 ↔ (3mm legnth) 4mm ID x 6mm OD Spacer:17
- [Mate]: RollerBearingShaft:33 ↔ 4x7x2.5mm Flanged Ball Bearing:67
- [Mate]: RollerBearingShaft:33 ↔ 4x7x2.5mm Flanged Ball Bearing:67
- [Mate]: 4x7x2.5mm Flanged Ball Bearing:66 ↔ RollerBearingShaft:33
- [Mate]: 4x7x2.5mm Flanged Ball Bearing:66 ↔ RollerBearingShaft:33
- [Mate]: (1mm legnth) 4mm ID x 6mm OD Spacer:34 ↔ 4x7x2.5mm Flanged Ball Bearing:66
- [Mate]: (1mm legnth) 4mm ID x 6mm OD Spacer:34 ↔ 4x7x2.5mm Flanged Ball Bearing:66
- [Mate]: (1mm legnth) 4mm ID x 6mm OD Spacer:33 ↔ 4x7x2.5mm Flanged Ball Bearing:68
- Mate:345: HousingFaceInput:1 ↔ (1mm legnth) 4mm ID x 6mm OD Spacer:34
- Mate:346: HousingFaceInput:1 ↔ 4x7x2.5mm Flanged Ball Bearing:68
- [Mate]: (1mm legnth) 4mm ID x 6mm OD Spacer:35 ↔ 4x7x2.5mm Flanged Ball Bearing:72
- [Mate]: 4x7x2.5mm Flanged Ball Bearing:72 ↔ RollerBearingShaft:36
- [Mate]: 4x7x2.5mm Flanged Ball Bearing:72 ↔ RollerBearingShaft:36
- [Mate]: RollerBearingShaft:36 ↔ 4x7x2.5mm Flanged Ball Bearing:73
- [Mate]: RollerBearingShaft:36 ↔ 4x7x2.5mm Flanged Ball Bearing:73
- [Mate]: 4x7x2.5mm Flanged Ball Bearing:73 ↔ (3mm legnth) 4mm ID x 6mm OD Spacer:18
- [Mate]: 4x7x2.5mm Flanged Ball Bearing:73 ↔ (3mm legnth) 4mm ID x 6mm OD Spacer:18
- [Mate]: 4x7x2.5mm Flanged Ball Bearing:71 ↔ (3mm legnth) 4mm ID x 6mm OD Spacer:18
- [Mate]: 4x7x2.5mm Flanged Ball Bearing:71 ↔ (3mm legnth) 4mm ID x 6mm OD Spacer:18
- [Mate]: RollerBearingShaft:35 ↔ 4x7x2.5mm Flanged Ball Bearing:71
- [Mate]: RollerBearingShaft:35 ↔ 4x7x2.5mm Flanged Ball Bearing:71
- [Mate]: 4x7x2.5mm Flanged Ball Bearing:70 ↔ RollerBearingShaft:35
- [Mate]: 4x7x2.5mm Flanged Ball Bearing:70 ↔ RollerBearingShaft:35
- [Mate]: (1mm legnth) 4mm ID x 6mm OD Spacer:36 ↔ 4x7x2.5mm Flanged Ball Bearing:70
- [Mate]: (1mm legnth) 4mm ID x 6mm OD Spacer:36 ↔ 4x7x2.5mm Flanged Ball Bearing:70
- [Mate]: (1mm legnth) 4mm ID x 6mm OD Spacer:35 ↔ 4x7x2.5mm Flanged Ball Bearing:72
- Mate:363: HousingFaceInput:1 ↔ (1mm legnth) 4mm ID x 6mm OD Spacer:36
- Mate:364: HousingFaceInput:1 ↔ 4x7x2.5mm Flanged Ball Bearing:72
- Mate:365: 4x7x2.5mm Flanged Ball Bearing:22 ↔ CycloidalDisk:1
- Tangent:1: 4x7x2.5mm Flanged Ball Bearing:22 ↔ CycloidalDisk:1
- Mate:366: 4x7x2.5mm Flanged Ball Bearing:25 ↔ CycloidalDisk:2
- Flush:1: CycloidalDisk:2 ↔ 16mm ID x 22mm OD x 4mm Thickness Ball Bearing:1
- Mate:367: CycloidalDisk:2 ↔ 16mm ID x 22mm OD x 4mm Thickness Ball Bearing:1
- Flush:2: CycloidalDisk:1 ↔ 16mm ID x 22mm OD x 4mm Thickness Ball Bearing:2
- Mate:368: CycloidalDisk:1 ↔ 16mm ID x 22mm OD x 4mm Thickness Ball Bearing:2
- Flush:3: 16mm ID x 22mm OD x 4mm Thickness Ball Bearing:2 ↔ EccentricBearingShaft:1
- Mate:369: 16mm ID x 22mm OD x 4mm Thickness Ball Bearing:2 ↔ EccentricBearingShaft:1
- Mate:370: 16mm ID x 22mm OD x 4mm Thickness Ball Bearing:1 ↔ EccentricBearingShaft:1
- Tangent:2: 4x7x2.5mm Flanged Ball Bearing:7 ↔ CycloidalDisk:1
- Tangent:3: 4x7x2.5mm Flanged Ball Bearing:16 ↔ CycloidalDisk:2
- Tangent:4: 4x7x2.5mm Flanged Ball Bearing:68 ↔ CycloidalDisk:2
## Named parameters: d439_d394 = 0 mm, d440_d349 = 0 mm, d441_d350 = 0 mm, d442_d351 = 0 mm, d443_d352 = 0 mm, d444_d353 = 0 mm, d445_d354 = 0 mm, d446_d355 = 0 mm, d447_d340 = 0 mm, d448_d342 = 0 mm, d449_d343 = 0 mm, d450_d344 = 0 mm, d451_d345 = 0 mm, d452_d346 = 0 mm, d453_d347 = 0 mm, d454_d348 = 0 mm, d457_d394 = 0 mm, d458_d349 = 0 mm, d459_d350 = 0 mm, d460_d351 = 0 mm, d461_d352 = 0 mm, d462_d353 = 0 mm, d463_d354 = 0 mm, d464_d355 = 0 mm, d465_d340 = 0 mm, d466_d342 = 0 mm, d467_d343 = 0 mm, d468_d344 = 0 mm, d469_d345 = 0 mm, d470_d346 = 0 mm, d471_d347 = 0 mm, d472_d348 = 0 mm, d475_d394 = 0 mm, d476_d349 = 0 mm, d477_d350 = 0 mm, d478_d351 = 0 mm, d479_d352 = 0 mm, d480_d353 = 0 mm, d481_d354 = 0 mm, d482_d355 = 0 mm, d483_d340 = 0 mm, d484_d342 = 0 mm, d485_d343 = 0 mm, d486_d344 = 0 mm, d487_d345 = 0 mm, d488_d346 = 0 mm, d489_d347 = 0 mm, d490_d348 = 0 mm, d493_d394 = 0 mm, d494_d349 = 0 mm, d495_d350 = 0 mm, d496_d351 = 0 mm, d497_d352 = 0 mm, d498_d353 = 0 mm, d499_d354 = 0 mm, d500_d355 = 0 mm, d501_d340 = 0 mm, d502_d342 = 0 mm, d503_d343 = 0 mm, d504_d344 = 0 mm, d505_d345 = 0 mm, d506_d346 = 0 mm, d507_d347 = 0 mm, d508_d348 = 0 mm, d511_d394 = 0 mm, d512_d349 = 0 mm, d513_d350 = 0 mm, d514_d351 = 0 mm, d515_d352 = 0 mm, d516_d353 = 0 mm, d517_d354 = 0 mm, d518_d355 = 0 mm, d519_d340 = 0 mm, d520_d342 = 0 mm, d521_d343 = 0 mm, d522_d344 = 0 mm, d523_d345 = 0 mm, d524_d346 = 0 mm, d525_d347 = 0 mm, d526_d348 = 0 mm, d529_d394 = 0 mm, d530_d349 = 0 mm, d531_d350 = 0 mm, d532_d351 = 0 mm, d533_d352 = 0 mm, d534_d353 = 0 mm, d535_d354 = 0 mm, d536_d355 = 0 mm, d537_d340 = 0 mm, d538_d342 = 0 mm, d539_d343 = 0 mm, d540_d344 = 0 mm, d541_d345 = 0 mm, d542_d346 = 0 mm, d543_d347 = 0 mm, d544_d348 = 0 mm, d547_d394 = 0 mm, d548_d349 = 0 mm, d549_d350 = 0 mm, d550_d351 = 0 mm, d551_d352 = 0 mm, d552_d353 = 0 mm, d553_d354 = 0 mm, d554_d355 = 0 mm, d555_d340 = 0 mm, d556_d342 = 0 mm, d557_d343 = 0 mm, d558_d344 = 0 mm, d559_d345 = 0 mm, d560_d346 = 0 mm, d561_d347 = 0 mm, d562_d348 = 0 mm, d565_d394 = 0 mm, d566_d349 = 0 mm, d567_d350 = 0 mm, d568_d351 = 0 mm, d569_d352 = 0 mm, d570_d353 = 0 mm, d571_d354 = 0 mm, d572_d355 = 0 mm, d573_d340 = 0 mm, d574_d342 = 0 mm, d575_d343 = 0 mm, d576_d344 = 0 mm, d577_d345 = 0 mm, d578_d346 = 0 mm, d579_d347 = 0 mm, d580_d348 = 0 mm, d583_d394 = 0 mm, d584_d349 = 0 mm, d585_d350 = 0 mm, d586_d351 = 0 mm, d587_d352 = 0 mm, d588_d353 = 0 mm, d589_d354 = 0 mm, d590_d355 = 0 mm, d591_d340 = 0 mm, d592_d342 = 0 mm, d593_d343 = 0 mm, d594_d344 = 0 mm, d595_d345 = 0 mm, d596_d346 = 0 mm, d597_d347 = 0 mm, d598_d348 = 0 mm, d601_d394 = 0 mm, d602_d349 = 0 mm, d603_d350 = 0 mm, d604_d351 = 0 mm, d605_d352 = 0 mm, d606_d353 = 0 mm, d607_d354 = 0 mm, d608_d355 = 0 mm, d609_d340 = 0 mm, d610_d342 = 0 mm, d611_d343 = 0 mm, d612_d344 = 0 mm, d613_d345 = 0 mm, d614_d346 = 0 mm, d615_d347 = 0 mm, d616_d348 = 0 mm, d619_d394 = 0 mm, d620_d349 = 0 mm, d621_d350 = 0 mm, d622_d351 = 0 mm, d623_d352 = 0 mm, d624_d353 = 0 mm, d625_d354 = 0 mm, d626_d355 = 0 mm, d627_d340 = 0 mm, d628_d342 = 0 mm, d629_d343 = 0 mm, d630_d344 = 0 mm, d631_d345 = 0 mm, d632_d346 = 0 mm, d633_d347 = 0 mm, d634_d348 = 0 mm, d637_d394 = 0 mm, d638_d349 = 0 mm, d639_d350 = 0 mm, d640_d351 = 0 mm, d641_d352 = 0 mm, d642_d353 = 0 mm, d643_d354 = 0 mm, d644_d355 = 0 mm, d645_d340 = 0 mm, d646_d342 = 0 mm, d647_d343 = 0 mm, d648_d344 = 0 mm, d649_d345 = 0 mm, d650_d346 = 0 mm, d651_d347 = 0 mm, d652_d348 = 0 mm, d655_d394 = 0 mm, d656_d349 = 0 mm, d657_d350 = 0 mm, d658_d351 = 0 mm, d659_d352 = 0 mm, d660_d353 = 0 mm, d661_d354 = 0 mm, d662_d355 = 0 mm, d663_d340 = 0 mm, d664_d342 = 0 mm, d665_d343 = 0 mm, d666_d344 = 0 mm, d667_d345 = 0 mm, d668_d346 = 0 mm, d669_d347 = 0 mm, d670_d348 = 0 mm, d673_d394 = 0 mm, d674_d349 = 0 mm, d675_d350 = 0 mm, d676_d351 = 0 mm, d677_d352 = 0 mm, d678_d353 = 0 mm, d679_d354 = 0 mm, d680_d355 = 0 mm, d681_d340 = 0 mm, d682_d342 = 0 mm, d683_d343 = 0 mm, d684_d344 = 0 mm, d685_d345 = 0 mm, d686_d346 = 0 mm, d687_d347 = 0 mm, d688_d348 = 0 mm, d691_d394 = 0 mm, d692_d349 = 0 mm, d693_d350 = 0 mm, d694_d351 = 0 mm, d695_d352 = 0 mm, d696_d353 = 0 mm, d697_d354 = 0 mm, d698_d355 = 0 mm, d699_d340 = 0 mm, d700_d342 = 0 mm, d701_d343 = 0 mm, d702_d344 = 0 mm, d703_d345 = 0 mm, d704_d346 = 0 mm, d705_d347 = 0 mm, d706_d348 = 0 mm, d709_d394 = 0 mm, d710_d349 = 0 mm, d711_d350 = 0 mm, d712_d351 = 0 mm, d713_d352 = 0 mm, d714_d353 = 0 mm, d715_d354 = 0 mm, d716_d355 = 0 mm, d717_d340 = 0 mm, d718_d342 = 0 mm, d719_d343 = 0 mm, d720_d344 = 0 mm, d721_d345 = 0 mm, d722_d346 = 0 mm, d723_d347 = 0 mm, d724_d348 = 0 mm, d727_d394 = 0 mm, d728_d349 = 0 mm, d729_d350 = 0 mm, d730_d351 = 0 mm, d731_d352 = 0 mm, d732_d353 = 0 mm, d733_d354 = 0 mm, d734_d355 = 0 mm, d735_d340 = 0 mm, d736_d342 = 0 mm, d737_d343 = 0 mm, d738_d344 = 0 mm, d739_d345 = 0 mm, d740_d346 = 0 mm, d741_d347 = 0 mm, d742_d348 = 0 mm
